# Autodesk Inventor assembly: motor unit 2820
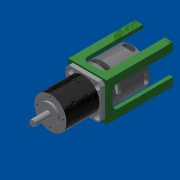
[picture p0: Inventor's stored thumbnail of the model, 180x180]
Saved by Autodesk Inventor 2018 (Build 220112000, 112)
## iProperties
Created: 2020-06-06
Part Number: motor unit 2820
Document SubType Name: Assembly
Designer: Bunny320
Author: Bunny320
## Documents named in this file (6)
- C:\Users\Bunny320\Desktop\sechs\4-CAD\motor unit 2820.iam
- C:\Users\Bunny320\Desktop\sechs\4-CAD\921-2820 house.ipt
- C:\Users\Bunny320\Desktop\sechs\4-CAD\standardParts\AS 2820 kv880\AS 2820 kv880.ipt
- C:\Users\Bunny320\Desktop\sechs\4-CAD\912-35-reducer.ipt
- C:\Users\Bunny320\Desktop\sechs\4-CAD\922-2820 magnet hold.ipt
- C:\Users\Bunny320\Desktop\sechs\4-CAD\magnet-4x4.ipt
## Components (5 placed, 5 different names)
1. 921-2820 house:1 — Flush:1, Flush:2, Flush:3, Mate:1, Mate:2, Mate:3, Mate:4, Mate:5, Mate:6
2. AS 2820 kv880:1 — Mate:4, Mate:5, Mate:6, Mate:7, Mate:8, Mate:9
3. 912-35-reducer:1 — Mate:1, Mate:2, Mate:3
4. 922-2820 magnet hold:1 — Mate:7, Mate:8, Mate:9, Mate:10, Mate:11
5. magnet-4x4:1 — Mate:10, Mate:11
## Relationships (14: Mate 11, Flush 3)
- Flush:1: 921-2820 house:1
- Flush:2: 921-2820 house:1
- Flush:3: 921-2820 house:1
- Mate:1: 921-2820 house:1 ↔ 912-35-reducer:1
- Mate:2: 921-2820 house:1 ↔ 912-35-reducer:1
- Mate:3: 921-2820 house:1 ↔ 912-35-reducer:1
- Mate:4: 921-2820 house:1 ↔ AS 2820 kv880:1
- Mate:5: 921-2820 house:1 ↔ AS 2820 kv880:1
- Mate:6: 921-2820 house:1 ↔ AS 2820 kv880:1
- Mate:7: AS 2820 kv880:1 ↔ 922-2820 magnet hold:1
- Mate:8: AS 2820 kv880:1 ↔ 922-2820 magnet hold:1
- Mate:9: AS 2820 kv880:1 ↔ 922-2820 magnet hold:1
- Mate:10: 922-2820 magnet hold:1 ↔ magnet-4x4:1
- Mate:11: 922-2820 magnet hold:1 ↔ magnet-4x4:1
